# Autodesk Inventor assembly: use this - gimme that tech award
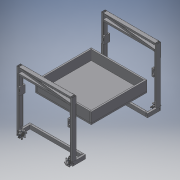
[picture p0: Inventor's stored thumbnail of the model, 180x180]
Saved by Autodesk Inventor 2018 (Build 220112000, 112)
## iProperties
Created: 2019-01-10
Part Number: use this - gimme that tech award
Document SubType Name: Assembly
Designer: maste
Author: maste
## Documents named in this file (4)
- \\studenthome\students\S-2512711\GitHub\2019CAD\Drivebase but Calvin is a mad man\use this - gimme that tech award.iam
- \\studenthome\students\S-2512711\GitHub\2019CAD\Drivebase but Calvin is a mad man\Slidey Mecanum L thing V2.iam
- \\studenthome\students\S-2512711\GitHub\2019CAD\Drivebase but Calvin is a mad man\Temporary Guide.ipt
- \\studenthome\students\S-2512711\GitHub\2019CAD\Drivebase but Calvin is a mad man\Platform.iam
## Components (7 placed, 3 different names)
1. Slidey Mecanum L thing V2:1 [sub-assembly] — Mate:17, Flush:16, Mate:18, Flush:17
2. Slidey Mecanum L thing V2:2 [sub-assembly] — Mate:19, Flush:18, Mate:20, Flush:19
3. Temporary Guide:1 — Mate:20, Flush:19
4. Temporary Guide:2 — Mate:18, Flush:17
5. Temporary Guide:3 — Mate:17, Flush:16
6. Temporary Guide:4 — Mate:19, Flush:18
7. Platform:1 [sub-assembly]
## Relationships (8: Mate 4, Flush 4)
- Mate:17: Slidey Mecanum L thing V2:1 ↔ Temporary Guide:3
- Flush:16 (-16.9164 mm): Slidey Mecanum L thing V2:1 ↔ Temporary Guide:3
- Mate:18: Slidey Mecanum L thing V2:1 ↔ Temporary Guide:2
- Flush:17 (-16.9164 mm): Slidey Mecanum L thing V2:1 ↔ Temporary Guide:2
- Mate:19: Slidey Mecanum L thing V2:2 ↔ Temporary Guide:4
- Flush:18 (-16.9164 mm): Slidey Mecanum L thing V2:2 ↔ Temporary Guide:4
- Mate:20: Slidey Mecanum L thing V2:2 ↔ Temporary Guide:1
- Flush:19 (-16.9164 mm): Slidey Mecanum L thing V2:2 ↔ Temporary Guide:1
